# Autodesk Inventor assembly: 3_25_Omni-Directional_Wheel_276-3526
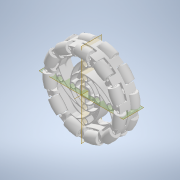
[picture p0: Inventor's stored thumbnail of the model, 180x180]
Saved by Autodesk Inventor 2020 (Build 240168000, 168)
## iProperties
Created: 2014-01-09
Part Number: 3_25_Omni-Directional_Wheel_276-3526
Description: STEP AP203
Document SubType Name: Assembly
Designer: Alex Zaccardelli
Sending System: SolidWorks 2013
Preprocessor: SwSTEP 2.0
Title: 276-3526-000 rev 1.STEP
Revision Number: ANY
## Documents named in this file (3)
- D:\DR4BTrayBot\SIGBotsCADLibrary\3_25_Omni-Directional_Wheel_276-3526.iam
- D:\DR4BTrayBot\SIGBotsCADLibrary\276-3526-004 Rev 1.ipt
- D:\DR4BTrayBot\SIGBotsCADLibrary\Roller Assembly.iam
## Components (23 placed, 23 different names)
1. 276-3526-004 Rev 1_1 — Mate:1
2. Roller Assembly_2 [sub-assembly]
3. Roller Assembly_3 [sub-assembly]
4. Roller Assembly_4 [sub-assembly]
5. Roller Assembly_5 [sub-assembly]
6. Roller Assembly_6 [sub-assembly]
7. Roller Assembly_7 [sub-assembly]
8. Roller Assembly_8 [sub-assembly]
9. Roller Assembly_9 [sub-assembly]
10. Roller Assembly_10 [sub-assembly]
11. Roller Assembly_11 [sub-assembly]
12. Roller Assembly_12 [sub-assembly]
13. Roller Assembly_13 [sub-assembly]
14. Roller Assembly_14 [sub-assembly]
15. Roller Assembly_15 [sub-assembly]
16. Roller Assembly_16 [sub-assembly]
17. Roller Assembly_17 [sub-assembly]
18. Roller Assembly_18 [sub-assembly]
19. Roller Assembly_19 [sub-assembly]
20. Roller Assembly_20 [sub-assembly]
21. Roller Assembly_21 [sub-assembly]
22. Roller Assembly_22 [sub-assembly]
23. Roller Assembly_23 [sub-assembly]
## Relationships (1: Mate 1)
- Mate:1: 276-3526-004 Rev 1_1
